# Autodesk Inventor assembly: Assembly1
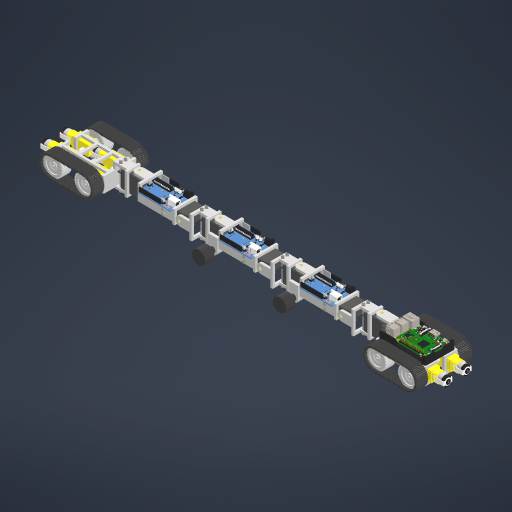
[picture p0: Inventor's stored thumbnail of the model, 512x512]
Saved by Autodesk Inventor 2024 (Build 280153000, 153)
## iProperties
Created: 2023-06-11
Part Number: Assembly1
Document SubType Name: Assembly
Designer: abhin
Author: abhin
## Documents named in this file (16)
- D:\Parth Folder\ES117\3D Model\Prototype 2\MBody(3).iam
- D:\Parth Folder\ES117\3D Model\Prototype 2\MG996R.ipt
- D:\Parth Folder\ES117\3D Model\Prototype 2\Sub Unit(1).ipt
- D:\Parth Folder\ES117\3D Model\Prototype 2\Wheel Holder.ipt
- D:\Parth Folder\ES117\3D Model\Prototype 2\Axis(1).ipt
- D:\Parth Folder\ES117\3D Model\Prototype 2\Small Wheels.ipt
- D:\Parth Folder\ES117\3D Model\Prototype 2\MHead(3).ipt
- D:\Parth Folder\ES117\3D Model\Prototype 2\MTail(3).ipt
- D:\Parth Folder\ES117\3D Model\Prototype 2\Sub Unit(2).ipt
- D:\Parth Folder\ES117\3D Model\Prototype 2\Bolt.ipt
- D:\Parth Folder\ES117\3D Model\Prototype 2\Nut.ipt
- D:\Parth Folder\ES117\3D Model\Prototype 2\BO DC Motor.iam
- D:\Parth Folder\ES117\3D Model\Prototype 2\Arduino\aurdino v5.iam
- D:\Parth Folder\ES117\3D Model\Prototype 2\Wheel.ipt
- D:\Parth Folder\ES117\3D Model\Prototype 2\Raspberry_Pi3\Raspberry_Pi4 v19.iam
- D:\Parth Folder\ES117\3D Model\Prototype 2\Track.ipt
## Components (75 placed, 15 different names)
1. MG996R:1 — Mate:1, Mate:38, Mate:39, Mate:152, Mate:153, Mate:161, Mate:162, Flush:43
2. Sub Unit(1):1 — Mate:1, Mate:3, Mate:4, Mate:38, Mate:39, Mate:54, Mate:55, Mate:68, Mate:69, Mate:74, Mate:75
3. MG996R:2 — Mate:3, Mate:4, Mate:45, Mate:46, Mate:47
4. MG996R:3 — Mate:17, Mate:18, Flush:6, Mate:32, Mate:33, Mate:34, Mate:48, Mate:49
5. Sub Unit(1):3 — Mate:13, Mate:14, Mate:32, Mate:33, Mate:34, Mate:52, Mate:53, Mate:64, Mate:65, Mate:86, Mate:87
6. MG996R:4 — Mate:13, Mate:14, Mate:40, Mate:41, Mate:42
7. MG996R:5 — Mate:26, Mate:28, Mate:43, Mate:44, Mate:165
8. Wheel Holder:1 — Mate:17, Mate:18, Mate:19, Flush:5, Flush:6
9. Axis(1):1 — Mate:19, Flush:5, Mate:20, Mate:21, Mate:22, Mate:23
10. Small Wheels:1 — Mate:21, Mate:22
11. Small Wheels:2 — Mate:20, Mate:23
12. MHead(3):1 — Mate:97, Mate:98, Mate:99, Mate:101, Mate:102, Mate:118, Mate:119, Flush:30, Flush:32, Mate:120, Mate:121, Flush:36, Mate:163, Mate:164
13. MTail(3):1 — Mate:26, Mate:28, Mate:60, Mate:61, Mate:90, Mate:91, Mate:92, Mate:94, Mate:95, Mate:111, Mate:113, Flush:25, Flush:39, Mate:165
14. Sub Unit(2):1 — Mate:40, Mate:41, Mate:42, Mate:43, Mate:44, Mate:58, Mate:59, Mate:62, Mate:63, Mate:78, Mate:79, Mate:124, Mate:125, Flush:38
15. Sub Unit(2):2 — Mate:45, Mate:46, Mate:47, Mate:48, Mate:49, Mate:56, Mate:57, Mate:66, Mate:67, Mate:70, Mate:71, Mate:122, Mate:123, Flush:37
16. Bolt:1 — Mate:60, Mate:84
17. Bolt:2 — Mate:61, Mate:85
18. Bolt:3 — Mate:52, Mate:64, Mate:89
19. Bolt:4 — Mate:53, Mate:65, Mate:88
20. Bolt:5 — Mate:55, Mate:68, Mate:77
21. Bolt:6 — Mate:54, Mate:69, Mate:76
22. Bolt:7 — Mate:56, Mate:67, Mate:73
23. Bolt:8 — Mate:57, Mate:66, Mate:72
24. Bolt:9 — Mate:59, Mate:62, Mate:81
25. Bolt:10 — Mate:58, Mate:63, Mate:80
26. Nut:1 — Mate:79, Mate:80
27. Nut:2 — Mate:78, Mate:81
28. Nut:3 — Mate:70, Mate:72
29. Nut:4 — Mate:71, Mate:73
30. Nut:5 — Mate:84
31. Nut:6 — Mate:85
32. Nut:7 — Mate:87, Mate:88
33. Nut:8 — Mate:86, Mate:89
34. Nut:9 — Mate:74, Mate:76
35. Nut:10 — Mate:75, Mate:77
36. BO DC Motor:1 [sub-assembly] — Mate:90, Mate:91, Mate:92, Mate:93, Flush:7, Flush:8, Flush:9, Mate:109
37. BO DC Motor:2 [sub-assembly] — Mate:93, Flush:7, Flush:8, Flush:10, Mate:108
38. BO DC Motor:3 [sub-assembly] — Mate:94, Flush:9, Mate:95, Mate:96, Flush:11, Mate:112
39. BO DC Motor:4 [sub-assembly] — Mate:96, Flush:10, Flush:11, Mate:110
40. BO DC Motor:5 [sub-assembly] — Mate:97, Mate:98, Mate:99, Mate:100, Flush:12, Flush:13, Flush:14, Mate:114
41. BO DC Motor:6 [sub-assembly] — Mate:101, Flush:14, Mate:102, Mate:103, Flush:16, Mate:116
42. BO DC Motor:7 [sub-assembly] — Mate:103, Flush:15, Flush:16, Mate:117
43. BO DC Motor:8 [sub-assembly] — Mate:100, Flush:12, Flush:13, Flush:15, Mate:115
44. Wheel:1 — Mate:108, Mate:111, Flush:19, Flush:24
45. Wheel:2 — Mate:109, Flush:19
46. Wheel:3 — Mate:114, Flush:21, Flush:31
47. Wheel:4 — Mate:115, Mate:118, Flush:21
48. Wheel:5 — Mate:117, Mate:119, Flush:22, Flush:33
49. Wheel:6 — Mate:116, Flush:22
50. Wheel:7 — Mate:112, Flush:20
51. Wheel:8 — Mate:110, Mate:113, Flush:20, Flush:27
52. Track:1 — Flush:24, Flush:25, Flush:28, Flush:29, Flush:40
53. Track:2 — Flush:27, Flush:28, Flush:29, Flush:39, Flush:40
54. Track:3 — Flush:33, Flush:34, Flush:35
55. Track:4 — Flush:30, Flush:31, Flush:32, Flush:34, Flush:35
56. Raspberry_Pi4 v19:1 [sub-assembly] — Mate:120, Mate:121, Flush:36
57. aurdino v5:1 [sub-assembly] — Mate:122, Mate:123, Flush:37
58. aurdino v5:2 [sub-assembly] — Mate:124, Mate:125, Flush:38
59. MG996R:6 — Mate:163, Mate:164
60. Sub Unit(1):4
61. MG996R:7
62. Sub Unit(2):3 — Mate:152, Mate:153
63. Bolt:11
64. Bolt:12
65. Bolt:13
66. Bolt:14
67. Nut:11
68. Nut:12
69. Nut:13
70. Nut:14
71. aurdino v5:3 [sub-assembly]
72. Wheel Holder:2 — Mate:161, Mate:162, Flush:43
73. Axis(1):2
74. Small Wheels:3
75. Small Wheels:4
## Relationships (170: Mate 135, Flush 35)
- Mate:1: MG996R:1 ↔ Sub Unit(1):1
- Mate:3: Sub Unit(1):1 ↔ MG996R:2
- Mate:4: Sub Unit(1):1 ↔ MG996R:2
- Mate:13: Sub Unit(1):3 ↔ MG996R:4
- Mate:14: Sub Unit(1):3 ↔ MG996R:4
- Mate:17: MG996R:3 ↔ Wheel Holder:1
- Mate:18: MG996R:3 ↔ Wheel Holder:1
- Mate:19: Wheel Holder:1 ↔ Axis(1):1
- Flush:5 (-25 mm): Wheel Holder:1 ↔ Axis(1):1
- Mate:20: Axis(1):1 ↔ Small Wheels:2
- Mate:21: Axis(1):1 ↔ Small Wheels:1
- Flush:6: MG996R:3 ↔ Wheel Holder:1
- Mate:22: Axis(1):1 ↔ Small Wheels:1
- Mate:23: Axis(1):1 ↔ Small Wheels:2
- Mate:26: MG996R:5 ↔ MTail(3):1
- Mate:28: MG996R:5 ↔ MTail(3):1
- Mate:32: MG996R:3 ↔ Sub Unit(1):3
- Mate:33: MG996R:3 ↔ Sub Unit(1):3
- Mate:34: MG996R:3 ↔ Sub Unit(1):3
- Mate:38: MG996R:1 ↔ Sub Unit(1):1
- Mate:39: MG996R:1 ↔ Sub Unit(1):1
- Mate:40: MG996R:4 ↔ Sub Unit(2):1
- Mate:41: MG996R:4 ↔ Sub Unit(2):1
- Mate:42: MG996R:4 ↔ Sub Unit(2):1
- Mate:43: MG996R:5 ↔ Sub Unit(2):1
- Mate:44: MG996R:5 ↔ Sub Unit(2):1
- Mate:45: MG996R:2 ↔ Sub Unit(2):2
- Mate:46: MG996R:2 ↔ Sub Unit(2):2
- Mate:47: MG996R:2 ↔ Sub Unit(2):2
- Mate:48: MG996R:3 ↔ Sub Unit(2):2
- Mate:49: MG996R:3 ↔ Sub Unit(2):2
- Mate:52: Sub Unit(1):3 ↔ Bolt:3
- Mate:53: Sub Unit(1):3 ↔ Bolt:4
- Mate:54: Sub Unit(1):1 ↔ Bolt:6
- Mate:55: Sub Unit(1):1 ↔ Bolt:5
- Mate:56: Sub Unit(2):2 ↔ Bolt:7
- Mate:57: Sub Unit(2):2 ↔ Bolt:8
- Mate:58: Sub Unit(2):1 ↔ Bolt:10
- Mate:59: Sub Unit(2):1 ↔ Bolt:9
- Mate:60: MTail(3):1 ↔ Bolt:1
- Mate:61: MTail(3):1 ↔ Bolt:2
- Mate:62: Sub Unit(2):1 ↔ Bolt:9
- Mate:63: Sub Unit(2):1 ↔ Bolt:10
- Mate:64: Sub Unit(1):3 ↔ Bolt:3
- Mate:65: Sub Unit(1):3 ↔ Bolt:4
- Mate:66: Sub Unit(2):2 ↔ Bolt:8
- Mate:67: Sub Unit(2):2 ↔ Bolt:7
- Mate:68: Sub Unit(1):1 ↔ Bolt:5
- Mate:69: Sub Unit(1):1 ↔ Bolt:6
- Mate:70: Sub Unit(2):2 ↔ Nut:3
- Mate:71: Sub Unit(2):2 ↔ Nut:4
- Mate:72: Bolt:8 ↔ Nut:3
- Mate:73: Bolt:7 ↔ Nut:4
- Mate:74: Sub Unit(1):1 ↔ Nut:9
- Mate:75: Sub Unit(1):1 ↔ Nut:10
- Mate:76: Bolt:6 ↔ Nut:9
- Mate:77: Bolt:5 ↔ Nut:10
- Mate:78: Sub Unit(2):1 ↔ Nut:2
- Mate:79: Sub Unit(2):1 ↔ Nut:1
- Mate:80: Bolt:10 ↔ Nut:1
- Mate:81: Bolt:9 ↔ Nut:2
- Mate:84: Bolt:1 ↔ Nut:5
- Mate:85: Bolt:2 ↔ Nut:6
- Mate:86: Sub Unit(1):3 ↔ Nut:8
- Mate:87: Sub Unit(1):3 ↔ Nut:7
- Mate:88: Bolt:4 ↔ Nut:7
- Mate:89: Bolt:3 ↔ Nut:8
- Mate:90: MTail(3):1 ↔ BO DC Motor:1
- Mate:91: MTail(3):1 ↔ BO DC Motor:1
- Mate:92: MTail(3):1 ↔ BO DC Motor:1
- Mate:93: BO DC Motor:1 ↔ BO DC Motor:2
- Flush:7: BO DC Motor:1 ↔ BO DC Motor:2
- Flush:8: BO DC Motor:1 ↔ BO DC Motor:2
- Mate:94: MTail(3):1 ↔ BO DC Motor:3
- Flush:9: BO DC Motor:1 ↔ BO DC Motor:3
- Mate:95: MTail(3):1 ↔ BO DC Motor:3
- Mate:96: BO DC Motor:3 ↔ BO DC Motor:4
- Flush:10: BO DC Motor:2 ↔ BO DC Motor:4
- Flush:11: BO DC Motor:3 ↔ BO DC Motor:4
- Mate:97: MHead(3):1 ↔ BO DC Motor:5
- Mate:98: MHead(3):1 ↔ BO DC Motor:5
- Mate:99: MHead(3):1 ↔ BO DC Motor:5
- Mate:100: BO DC Motor:5 ↔ BO DC Motor:8
- Flush:12: BO DC Motor:5 ↔ BO DC Motor:8
- Flush:13: BO DC Motor:5 ↔ BO DC Motor:8
- Mate:101: MHead(3):1 ↔ BO DC Motor:6
- Flush:14: BO DC Motor:5 ↔ BO DC Motor:6
- Mate:102: MHead(3):1 ↔ BO DC Motor:6
- Mate:103: BO DC Motor:6 ↔ BO DC Motor:7
- Flush:15: BO DC Motor:7 ↔ BO DC Motor:8
- Flush:16: BO DC Motor:6 ↔ BO DC Motor:7
- Mate:108: BO DC Motor:2 ↔ Wheel:1
- Mate:109: BO DC Motor:1 ↔ Wheel:2
- Mate:110: BO DC Motor:4 ↔ Wheel:8
- Mate:111: MTail(3):1 ↔ Wheel:1
- Flush:19: Wheel:1 ↔ Wheel:2
- Mate:112: BO DC Motor:3 ↔ Wheel:7
- Mate:113: MTail(3):1 ↔ Wheel:8
- Flush:20: Wheel:7 ↔ Wheel:8
- Mate:114: BO DC Motor:5 ↔ Wheel:3
- Mate:115: BO DC Motor:8 ↔ Wheel:4
- Mate:116: BO DC Motor:6 ↔ Wheel:6
- Mate:117: BO DC Motor:7 ↔ Wheel:5
- Mate:118: MHead(3):1 ↔ Wheel:4
- Mate:119: MHead(3):1 ↔ Wheel:5
- Flush:21: Wheel:3 ↔ Wheel:4
- Flush:22: Wheel:5 ↔ Wheel:6
- Flush:24: Wheel:1 ↔ Track:1
- Flush:25 (-2 mm): MTail(3):1 ↔ Track:1
- Flush:27: Wheel:8 ↔ Track:2
- Flush:28: Track:1 ↔ Track:2
- Flush:29: Track:1 ↔ Track:2
- Flush:30 (-3 mm): MHead(3):1 ↔ Track:4
- Flush:31: Wheel:3 ↔ Track:4
- Flush:32 (-6 mm): MHead(3):1 ↔ Track:4
- Flush:33: Wheel:5 ↔ Track:3
- Flush:34: Track:3 ↔ Track:4
- Flush:35: Track:3 ↔ Track:4
- Mate:120: MHead(3):1 ↔ Raspberry_Pi4 v19:1
- Mate:121: MHead(3):1 ↔ Raspberry_Pi4 v19:1
- Flush:36 (3 mm): MHead(3):1 ↔ Raspberry_Pi4 v19:1
- Mate:122: Sub Unit(2):2 ↔ aurdino v5:1
- Mate:123: Sub Unit(2):2 ↔ aurdino v5:1
- Flush:37: Sub Unit(2):2 ↔ aurdino v5:1
- Mate:124: Sub Unit(2):1 ↔ aurdino v5:2
- Mate:125: Sub Unit(2):1 ↔ aurdino v5:2
- Flush:38: Sub Unit(2):1 ↔ aurdino v5:2
- Flush:39 (-6.5 mm): MTail(3):1 ↔ Track:2
- Flush:40: Track:1 ↔ Track:2
- [Mate]: MG996R:6 ↔ Sub Unit(1):4
- [Mate]: Sub Unit(1):4 ↔ MG996R:7
- [Mate]: Sub Unit(1):4 ↔ MG996R:7
- [Mate]: MG996R:6 ↔ Sub Unit(1):4
- [Mate]: MG996R:6 ↔ Sub Unit(1):4
- [Mate]: MG996R:7 ↔ Sub Unit(2):3
- [Mate]: MG996R:7 ↔ Sub Unit(2):3
- [Mate]: MG996R:7 ↔ Sub Unit(2):3
- [Mate]: Sub Unit(1):4 ↔ Bolt:12
- [Mate]: Sub Unit(1):4 ↔ Bolt:11
- [Mate]: Sub Unit(2):3 ↔ Bolt:13
- [Mate]: Sub Unit(2):3 ↔ Bolt:14
- [Mate]: Sub Unit(2):3 ↔ Bolt:14
- [Mate]: Sub Unit(2):3 ↔ Bolt:13
- [Mate]: Sub Unit(1):4 ↔ Bolt:11
- [Mate]: Sub Unit(1):4 ↔ Bolt:12
- [Mate]: Sub Unit(2):3 ↔ Nut:11
- [Mate]: Sub Unit(2):3 ↔ Nut:12
- [Mate]: Bolt:14 ↔ Nut:11
- [Mate]: Bolt:13 ↔ Nut:12
- [Mate]: Sub Unit(1):4 ↔ Nut:13
- [Mate]: Sub Unit(1):4 ↔ Nut:14
- [Mate]: Bolt:12 ↔ Nut:13
- [Mate]: Bolt:11 ↔ Nut:14
- [Mate]: Sub Unit(2):3 ↔ aurdino v5:3
- [Mate]: Sub Unit(2):3 ↔ aurdino v5:3
- [Flush]: Sub Unit(2):3 ↔ aurdino v5:3
- Mate:152: MG996R:1 ↔ Sub Unit(2):3
- Mate:153: MG996R:1 ↔ Sub Unit(2):3
- [Mate]: Wheel Holder:2 ↔ Axis(1):2
- [Flush] (-25 mm): Wheel Holder:2 ↔ Axis(1):2
- [Mate]: Axis(1):2 ↔ Small Wheels:4
- [Mate]: Axis(1):2 ↔ Small Wheels:3
- [Mate]: Axis(1):2 ↔ Small Wheels:3
- [Mate]: Axis(1):2 ↔ Small Wheels:4
- Mate:161: MG996R:1 ↔ Wheel Holder:2
- Mate:162: MG996R:1 ↔ Wheel Holder:2
- Flush:43: MG996R:1 ↔ Wheel Holder:2
- Mate:163: MHead(3):1 ↔ MG996R:6
- Mate:164: MHead(3):1 ↔ MG996R:6
- Mate:165: MG996R:5 ↔ MTail(3):1
## Named parameters: d227_d190 = 0 mm, d228_d191 = 0 mm, d229_d192 = 0 mm, d230_d111 = 0 mm, d231_d112 = 0 mm, d232_d113 = 0 mm, d233_d81 = 0 mm, d234_d82 = 0 mm, d235_d83 = 0 mm, d236_d90 = 0 mm, d237_d91 = 0 mm, d238_d92 = 0 mm, d239_d93 = 0 mm, d240_d102 = 0 mm, d241_d103 = 0 mm, d242_d104 = 0 mm, d243_d105 = 0 mm, d244_d106 = 0 mm, d245_d107 = 0 mm, d246_d108 = 0 mm, d247_d109 = 0 mm, d248_d110 = 0 mm, d249_d74 = 0 mm, d250_d75 = 0 mm, d251_d0 = 0 mm, d252_d4 = 0 mm, d253_d5 = 0 mm, d258_d48 = 0 mm, d259_d49 = -25 mm, d260_d50 = 0 mm, d261_d51 = 0 mm, d262_d53 = 0 mm, d263_d54 = 0 mm
